# Autodesk Inventor assembly: LeggedBot
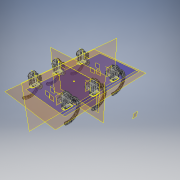
[picture p0: Inventor's stored thumbnail of the model, 180x180]
Saved by Autodesk Inventor 2016 (Build 200138000, 138)
## iProperties
Created: 2016-11-08
Part Number: LeggedBot
Document SubType Name: Assembly
Designer: brent
Author: brent
## Documents named in this file (4)
- C:\Users\brent\OneDrive\classes\desinv22\final\leggedbot_mechanical\LeggedBot.iam
- C:\Users\brent\OneDrive\classes\desinv22\final\leggedbot_mechanical\LegAssembly.iam
- C:\Users\brent\OneDrive\classes\desinv22\final\leggedbot_mechanical\LegAssembly_MIR.iam
- C:\Users\brent\OneDrive\classes\desinv22\final\leggedbot_mechanical\fabrication\Frame.ipt
## Components (7 placed, 3 different names)
1. LegAssembly:1 [sub-assembly] — Mate:1, Mate:9, Mate:18
2. LegAssembly:2 [sub-assembly] — Mate:8, Mate:11, Mate:20
3. LegAssembly:3 [sub-assembly] — Mate:7, Mate:10, Mate:19
4. LegAssembly_MIR:1 [sub-assembly] — Mate:17, Flush:11, Mate:18
5. LegAssembly_MIR:2 [sub-assembly] — Mate:16, Flush:10, Mate:19
6. LegAssembly_MIR:3 [sub-assembly] — Mate:15, Flush:9, Mate:20
7. Frame:1 — Flush:12
## Relationships (24: Flush 12, Mate 12)
- Flush:1 (115 mm)
- Flush:2 (-115 mm)
- Flush:3 (-88.9 mm)
- Flush:4 (101.6 mm)
- Mate:1: LegAssembly:1
- Mate:7 (-11 mm): LegAssembly:3
- Mate:8: LegAssembly:2
- Mate:9: LegAssembly:1
- Mate:10: LegAssembly:3
- Mate:11: LegAssembly:2
- Flush:5 (110 mm)
- Flush:6 (-110 mm)
- Flush:7 (110 mm)
- Flush:8 (-110 mm)
- Mate:15: LegAssembly_MIR:3
- Mate:16: LegAssembly_MIR:2
- Mate:17: LegAssembly_MIR:1
- Flush:9: LegAssembly_MIR:3
- Flush:10 (-11 mm): LegAssembly_MIR:2
- Flush:11: LegAssembly_MIR:1
- Mate:18: LegAssembly:1 ↔ LegAssembly_MIR:1
- Mate:19: LegAssembly:3 ↔ LegAssembly_MIR:2
- Mate:20: LegAssembly:2 ↔ LegAssembly_MIR:3
- Flush:12: Frame:1
